# Autodesk Inventor assembly: BHSS
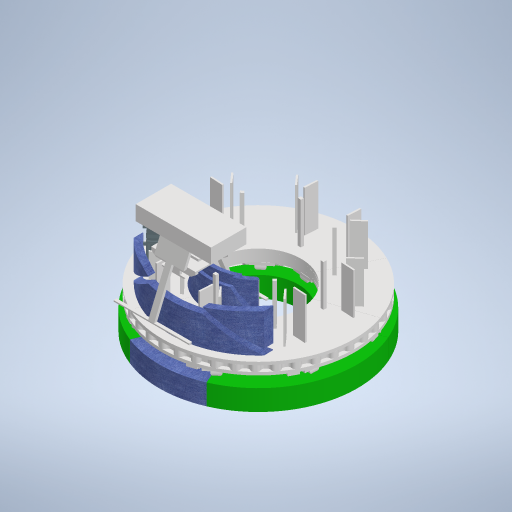
[picture p0: Inventor's stored thumbnail of the model, 512x512]
Saved by Autodesk Inventor 2023 (Build 270158000, 158)
## iProperties
Created: 2022-10-26
Part Number: BHSS
Document SubType Name: Assembly
Designer: cheng
Author: cheng
## Documents named in this file (10)
- C:\Users\cheng\Desktop\4th Year Project\Inventor\Third Assembly\Second Assembly\BHSS.iam
- C:\Users\cheng\Desktop\4th Year Project\Inventor\Third Assembly\Second Assembly\Battery Cage.ipt
- C:\Users\cheng\Desktop\4th Year Project\Inventor\Third Assembly\Second Assembly\Battery Container.ipt
- C:\Users\cheng\Desktop\4th Year Project\Inventor\Third Assembly\Second Assembly\Box Base Plate.ipt
- C:\Users\cheng\Desktop\4th Year Project\Inventor\Third Assembly\Second Assembly\Roller Carouel Assembly.iam
- C:\Users\cheng\Desktop\4th Year Project\Inventor\Third Assembly\Second Assembly\Carousel Fixed Track.ipt
- C:\Users\cheng\Desktop\4th Year Project\Inventor\Third Assembly\Second Assembly\Landing dock.ipt
- C:\Users\cheng\Desktop\4th Year Project\Inventor\Third Assembly\Second Assembly\drone model.ipt
- C:\Users\cheng\Desktop\4th Year Project\Inventor\Third Assembly\Second Assembly\Husky_3D_Model.ipt
- C:\Users\cheng\Desktop\4th Year Project\Inventor\Third Assembly\Second Assembly\Carousel Fixed Track Landing V3.ipt
## Components (23 placed, 9 different names)
1. Battery Cage:1 — Mate:77, Mate:78, Mate:103, Mate:104, Mate:105, Mate:106
2. Box Base Plate:1 — Mate:4, Mate:5, Mate:6, Mate:18, Mate:19, Mate:20, Mate:25, Flush:1, Mate:79, Mate:80, Mate:91
3. Carousel Fixed Track:1 — Mate:4, Mate:10, Mate:11, Mate:31, Mate:32, Mate:92, Mate:93
4. Carousel Fixed Track:2 — Mate:5, Mate:14, Mate:15, Mate:16, Mate:17
5. Carousel Fixed Track:3 — Mate:10, Mate:11, Mate:12, Mate:13, Mate:25, Mate:34, Mate:35, Mate:37, Mate:38, Mate:40, Mate:41, Mate:46, Mate:47
6. Carousel Fixed Track:4 — Mate:6, Mate:12, Mate:13, Mate:14, Mate:15, Mate:43, Mate:44
7. Carousel Fixed Track:5 — Mate:16, Mate:17, Mate:18, Mate:21, Mate:22
8. Carousel Fixed Track:6 — Mate:19, Mate:23, Mate:24, Mate:26, Mate:27
9. Carousel Fixed Track:7 — Mate:20, Mate:21, Mate:22, Mate:23, Mate:24
10. Roller Carouel Assembly:2 [sub-assembly] — Mate:31, Mate:32, Mate:33, Mate:36, Mate:87, Flush:9
11. Roller Carouel Assembly:3 [sub-assembly] — Mate:26, Mate:27, Mate:30
12. Roller Carouel Assembly:4 [sub-assembly] — Mate:34, Mate:35, Mate:36, Mate:39
13. Roller Carouel Assembly:5 [sub-assembly] — Mate:40, Mate:41, Mate:42, Mate:45
14. Roller Carouel Assembly:6 [sub-assembly] — Mate:46, Mate:47, Mate:48, Mate:97, Mate:98, Mate:101, Mate:102
15. Roller Carouel Assembly:7 [sub-assembly] — Mate:43, Mate:44, Mate:45, Mate:48
16. Roller Carouel Assembly:8 [sub-assembly] — Mate:37, Mate:38, Mate:39, Mate:42
17. Roller Carouel Assembly:9 [sub-assembly] — Mate:30, Mate:33, Mate:87, Flush:9
18. drone model:1 — Mate:77, Mate:78, Mate:103, Mate:104
19. Husky_3D_Model:1 — Flush:1
20. Landing dock:1 — Mate:79, Mate:80, Mate:105, Mate:106
21. Battery Container:18 — Mate:97, Mate:98
22. Carousel Fixed Track Landing V3:1 — Mate:91, Mate:92, Mate:93
23. Battery Container:19 — Mate:101, Mate:102
## Relationships (58: Mate 56, Flush 2)
- Mate:4: Box Base Plate:1 ↔ Carousel Fixed Track:1
- Mate:5: Box Base Plate:1 ↔ Carousel Fixed Track:2
- Mate:6: Box Base Plate:1 ↔ Carousel Fixed Track:4
- Mate:10: Carousel Fixed Track:1 ↔ Carousel Fixed Track:3
- Mate:11: Carousel Fixed Track:1 ↔ Carousel Fixed Track:3
- Mate:12: Carousel Fixed Track:3 ↔ Carousel Fixed Track:4
- Mate:13: Carousel Fixed Track:3 ↔ Carousel Fixed Track:4
- Mate:14: Carousel Fixed Track:2 ↔ Carousel Fixed Track:4
- Mate:15: Carousel Fixed Track:2 ↔ Carousel Fixed Track:4
- Mate:16: Carousel Fixed Track:2 ↔ Carousel Fixed Track:5
- Mate:17: Carousel Fixed Track:2 ↔ Carousel Fixed Track:5
- Mate:18: Box Base Plate:1 ↔ Carousel Fixed Track:5
- Mate:19: Box Base Plate:1 ↔ Carousel Fixed Track:6
- Mate:20: Box Base Plate:1 ↔ Carousel Fixed Track:7
- Mate:21: Carousel Fixed Track:5 ↔ Carousel Fixed Track:7
- Mate:22: Carousel Fixed Track:5 ↔ Carousel Fixed Track:7
- Mate:23: Carousel Fixed Track:6 ↔ Carousel Fixed Track:7
- Mate:24: Carousel Fixed Track:6 ↔ Carousel Fixed Track:7
- Mate:25: Box Base Plate:1 ↔ Carousel Fixed Track:3
- Mate:26: Carousel Fixed Track:6 ↔ Roller Carouel Assembly:3
- Mate:27: Carousel Fixed Track:6 ↔ Roller Carouel Assembly:3
- Mate:30: Roller Carouel Assembly:3 ↔ Roller Carouel Assembly:9
- Mate:31: Carousel Fixed Track:1 ↔ Roller Carouel Assembly:2
- Mate:32: Carousel Fixed Track:1 ↔ Roller Carouel Assembly:2
- Mate:33: Roller Carouel Assembly:2 ↔ Roller Carouel Assembly:9
- Mate:34: Carousel Fixed Track:3 ↔ Roller Carouel Assembly:4
- Mate:35: Carousel Fixed Track:3 ↔ Roller Carouel Assembly:4
- Mate:36: Roller Carouel Assembly:2 ↔ Roller Carouel Assembly:4
- Mate:37: Carousel Fixed Track:3 ↔ Roller Carouel Assembly:8
- Mate:38: Carousel Fixed Track:3 ↔ Roller Carouel Assembly:8
- Mate:39: Roller Carouel Assembly:4 ↔ Roller Carouel Assembly:8
- Mate:40: Carousel Fixed Track:3 ↔ Roller Carouel Assembly:5
- Mate:41: Carousel Fixed Track:3 ↔ Roller Carouel Assembly:5
- Mate:42: Roller Carouel Assembly:5 ↔ Roller Carouel Assembly:8
- Mate:43: Carousel Fixed Track:4 ↔ Roller Carouel Assembly:7
- Mate:44: Carousel Fixed Track:4 ↔ Roller Carouel Assembly:7
- Mate:45: Roller Carouel Assembly:5 ↔ Roller Carouel Assembly:7
- Mate:46: Carousel Fixed Track:3 ↔ Roller Carouel Assembly:6
- Mate:47: Carousel Fixed Track:3 ↔ Roller Carouel Assembly:6
- Mate:48: Roller Carouel Assembly:6 ↔ Roller Carouel Assembly:7
- Flush:1: Box Base Plate:1 ↔ Husky_3D_Model:1
- Mate:77: Battery Cage:1 ↔ drone model:1
- Mate:78: Battery Cage:1 ↔ drone model:1
- Mate:79: Box Base Plate:1 ↔ Landing dock:1
- Mate:80: Box Base Plate:1 ↔ Landing dock:1
- Mate:87: Roller Carouel Assembly:2 ↔ Roller Carouel Assembly:9
- Flush:9: Roller Carouel Assembly:2 ↔ Roller Carouel Assembly:9
- Mate:91: Box Base Plate:1 ↔ Carousel Fixed Track Landing V3:1
- Mate:92: Carousel Fixed Track:1 ↔ Carousel Fixed Track Landing V3:1
- Mate:93: Carousel Fixed Track:1 ↔ Carousel Fixed Track Landing V3:1
- Mate:97: Roller Carouel Assembly:6 ↔ Battery Container:18
- Mate:98: Roller Carouel Assembly:6 ↔ Battery Container:18
- Mate:101: Roller Carouel Assembly:6 ↔ Battery Container:19
- Mate:102: Roller Carouel Assembly:6 ↔ Battery Container:19
- Mate:103: Battery Cage:1 ↔ drone model:1
- Mate:104: Battery Cage:1 ↔ drone model:1
- Mate:105: Battery Cage:1 ↔ Landing dock:1
- Mate:106: Battery Cage:1 ↔ Landing dock:1
